# Autodesk Inventor assembly: 組合1
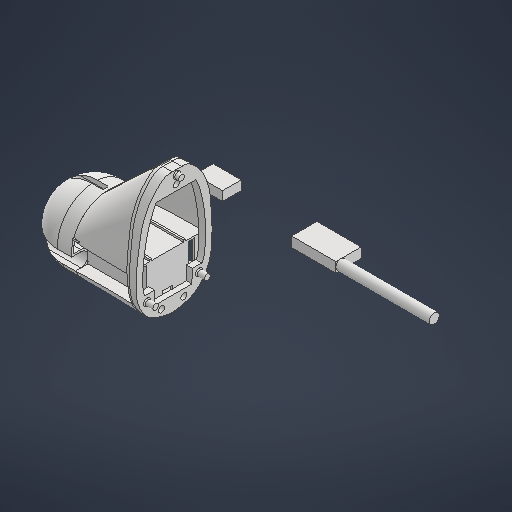
[picture p0: Inventor's stored thumbnail of the model, 512x512]
Saved by Autodesk Inventor 2026.2 (Build 302298000, 298)
## iProperties
Created: 2026-01-10
Part Number: 組合1
Document SubType Name: Assembly
Designer: gavin
Author: gavin
## Documents named in this file (6)
- D:\Inventor\skysurfer electric compartment\組合1.iam
- D:\Inventor\skysurfer electric compartment\baseplate.ipt
- D:\Inventor\skysurfer electric compartment\rc reciever.ipt
- D:\Inventor\skysurfer electric compartment\telementry.ipt
- D:\Inventor\skysurfer electric compartment\FC compartment.ipt
- D:\Inventor\skysurfer electric compartment\nosecone.ipt
## Components (5 placed, 5 different names)
1. baseplate:1 — 齊平:1
2. rc reciever:1
3. telementry:1
4. FC compartment:1 — 齊平:1, 剛性:1
5. nosecone:1 — 剛性:1
## Relationships (2: Flush 1, WeldJoint 1)
- 齊平:1 [Flush]: baseplate:1 ↔ FC compartment:1
- 剛性:1 [WeldJoint]: FC compartment:1 ↔ nosecone:1
